# Autodesk Inventor assembly: Shoulder_Pitch_Assembly
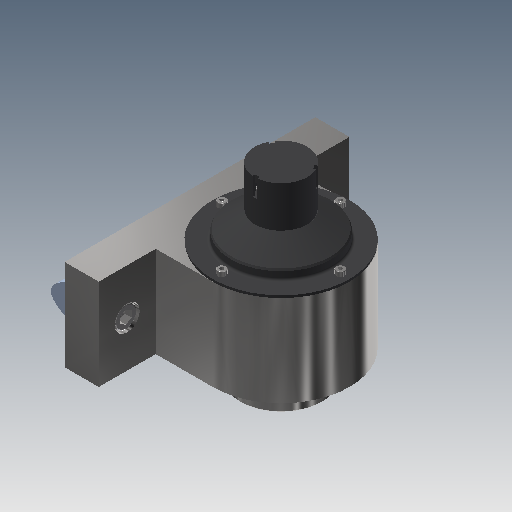
[picture p0: Inventor's stored thumbnail of the model, 512x512]
Saved by Autodesk Inventor 2021.4 (Build 254397000, 397)
## iProperties
Created: 2022-08-02
Part Number: Shoulder_Pitch_Assembly
Material: Generisch
Document SubType Name: Assembly
Designer: alexw
Mass: 1417.09 g
Surface Area: 710.967 cm^2
Volume: 192.324 cm^3
Density: 7.36827 g/cm^3
Author: alexw
## Documents named in this file (13)
- C:\Users\alexw\Documents\Inventor\Projects\03_CurrentProjects\MasterThesis\TrainingConsol_220422\Workgroups\Workgroup\Shoulder_Pitch_Assembly.iam
- C:\Users\alexw\Documents\Inventor\Projects\03_CurrentProjects\MasterThesis\TrainingConsol_220422\Workgroups\Workgroup\shoulder_joint_fit_v2.ipt
- C:\Users\alexw\Documents\Inventor\Projects\03_CurrentProjects\MasterThesis\TrainingConsol_220422\Workgroups\Workgroup\DIN 720 SKF - SKF 32005 X_Q.ipt
- C:\Users\alexw\Documents\Inventor\Projects\03_CurrentProjects\MasterThesis\TrainingConsol_220422\Workgroups\Workgroup\DIN 720 SKF - SKF 32004 X_Q.ipt
- C:\Users\alexw\Documents\Inventor\Projects\03_CurrentProjects\MasterThesis\TrainingConsol_220422\Workgroups\Workgroup\DIN EN ISO 7090 -  18.ipt
- C:\Users\alexw\Documents\Inventor\Projects\03_CurrentProjects\MasterThesis\TrainingConsol_220422\Workgroups\Workgroup\DIN 981 - KM 3.ipt
- C:\Users\alexw\Documents\Inventor\Projects\03_CurrentProjects\MasterThesis\TrainingConsol_220422\Workgroups\Workgroup\Shoulder_Shaft_Pitch.ipt
- C:\Users\alexw\Documents\Inventor\Projects\03_CurrentProjects\MasterThesis\TrainingConsol_220422\Workgroups\Workgroup\DIN EN ISO 4762 - M6 x 16.ipt
- C:\Users\alexw\Documents\Inventor\Projects\03_CurrentProjects\MasterThesis\TrainingConsol_220422\Workgroups\Workgroup\item_0038851_T-Slot_Nut_8_St_M6.ipt
- C:\Users\alexw\Documents\Inventor\Projects\03_CurrentProjects\MasterThesis\TrainingConsol_220422\Workgroups\Workgroup\Shoulder_Pitch_Sensor_Connector.ipt
- C:\Users\alexw\Documents\Inventor\Projects\03_CurrentProjects\MasterThesis\TrainingConsol_220422\Workgroups\Workgroup\Magnetic Encoder.ipt
- C:\Users\alexw\Documents\Inventor\Projects\03_CurrentProjects\MasterThesis\TrainingConsol_220422\Workgroups\Workgroup\DIN EN ISO 4762 - M2 x 8.ipt
- C:\Users\alexw\Documents\Inventor\Projects\03_CurrentProjects\MasterThesis\TrainingConsol_220422\Workgroups\Workgroup\DIN EN ISO 4762 - M2 x 6.ipt
## Components (18 placed, 12 different names)
1. shoulder_joint_fit_v2:1 — Mate:33, Flush:1, Mate:34, Mate:35, Angle:1, Angle:2
2. DIN 720 SKF- Präzision SKF 32005 X/Q:1
3. DIN 720 SKF- Präzision SKF 32004 X/Q:1
4. DIN EN ISO 7090 18:1
5. DIN 981 KM 3:1
6. Shoulder_Shaft_Pitch:1
7. DIN EN ISO 4762 M6 x 16:1 — Mate:37
8. DIN EN ISO 4762 M6 x 16:2 — Mate:36
9. Shoulder_Pitch_Sensor_Connector:1
10. Magnetic Encoder:1
11. DIN EN ISO 4762 M2 x 8:1
12. DIN EN ISO 4762 M2 x 8:2 — Mate:35
13. DIN EN ISO 4762 M2 x 8:3
14. DIN EN ISO 4762 M2 x 8:4
15. DIN EN ISO 4762 M2 x 6:1
16. DIN EN ISO 4762 M2 x 6:2
17. item_0038851_T-Slot_Nut_8_St_M6:1 — Mate:36, Angle:1, Flush:2
18. item_0038851_T-Slot_Nut_8_St_M6:2 — Mate:37, Angle:2, Flush:2
## Relationships (40: Mate 36, Flush 2, Angle 2)
- [Mate]: DIN 720 SKF- Präzision SKF 32004 X/Q:1 ↔ DIN EN ISO 7090 18:1
- [Mate]: DIN 720 SKF- Präzision SKF 32005 X/Q:1 ↔ Shoulder_Shaft_Pitch:1
- [Mate]: DIN EN ISO 7090 18:1 ↔ Shoulder_Shaft_Pitch:1
- [Mate]: DIN 981 KM 3:1 ↔ Shoulder_Shaft_Pitch:1
- [Mate]: DIN EN ISO 7090 18:1 ↔ DIN 981 KM 3:1
- [Mate]: shoulder_joint_fit_v2:1 ↔ Shoulder_Pitch_Sensor_Connector:1
- [Mate]: Shoulder_Pitch_Sensor_Connector:1 ↔ Magnetic Encoder:1
- [Mate]: Shoulder_Pitch_Sensor_Connector:1 ↔ DIN EN ISO 4762 M2 x 8:1
- [Mate]: Shoulder_Pitch_Sensor_Connector:1 ↔ DIN EN ISO 4762 M2 x 8:2
- [Mate]: Shoulder_Pitch_Sensor_Connector:1 ↔ DIN EN ISO 4762 M2 x 8:3
- [Mate]: Shoulder_Pitch_Sensor_Connector:1 ↔ DIN EN ISO 4762 M2 x 8:4
- [Mate]: Magnetic Encoder:1 ↔ DIN EN ISO 4762 M2 x 6:1
- [Mate]: Magnetic Encoder:1 ↔ DIN EN ISO 4762 M2 x 6:2
- [Mate]: DIN 720 SKF- Präzision SKF 32005 X/Q:1 ↔ Shoulder_Shaft_Pitch:1
- [Mate]: shoulder_joint_fit_v2:1 ↔ DIN EN ISO 4762 M6 x 16:2
- [Mate]: shoulder_joint_fit_v2:1 ↔ DIN EN ISO 4762 M6 x 16:2
- [Mate]: shoulder_joint_fit_v2:1 ↔ DIN EN ISO 4762 M6 x 16:1
- [Mate]: shoulder_joint_fit_v2:1 ↔ DIN EN ISO 4762 M6 x 16:1
- [Mate]: shoulder_joint_fit_v2:1 ↔ DIN 720 SKF- Präzision SKF 32005 X/Q:1
- [Mate]: DIN 720 SKF- Präzision SKF 32004 X/Q:1 ↔ Shoulder_Shaft_Pitch:1
- [Mate]: shoulder_joint_fit_v2:1 ↔ DIN 720 SKF- Präzision SKF 32004 X/Q:1
- [Mate]: shoulder_joint_fit_v2:1 ↔ Shoulder_Pitch_Sensor_Connector:1
- [Mate]: Shoulder_Pitch_Sensor_Connector:1 ↔ Magnetic Encoder:1
- [Mate]: shoulder_joint_fit_v2:1 ↔ Shoulder_Pitch_Sensor_Connector:1
- [Mate]: shoulder_joint_fit_v2:1 ↔ DIN EN ISO 4762 M2 x 8:1
- [Mate]: Shoulder_Pitch_Sensor_Connector:1 ↔ DIN EN ISO 4762 M2 x 8:4
- [Mate]: Shoulder_Pitch_Sensor_Connector:1 ↔ DIN EN ISO 4762 M2 x 8:3
- [Mate]: Shoulder_Pitch_Sensor_Connector:1 ↔ Magnetic Encoder:1
- [Mate]: Shoulder_Pitch_Sensor_Connector:1 ↔ DIN EN ISO 4762 M2 x 6:1
- [Mate]: Shoulder_Pitch_Sensor_Connector:1 ↔ DIN EN ISO 4762 M2 x 6:2
- [Mate]: shoulder_joint_fit_v2:1 ↔ Shoulder_Shaft_Pitch:1
- Mate:33: shoulder_joint_fit_v2:1
- Flush:1: shoulder_joint_fit_v2:1
- Mate:34: shoulder_joint_fit_v2:1
- Mate:35: shoulder_joint_fit_v2:1 ↔ DIN EN ISO 4762 M2 x 8:2
- Mate:36: DIN EN ISO 4762 M6 x 16:2 ↔ item_0038851_T-Slot_Nut_8_St_M6:1
- Angle:1 (0 deg): shoulder_joint_fit_v2:1 ↔ item_0038851_T-Slot_Nut_8_St_M6:1
- Mate:37: DIN EN ISO 4762 M6 x 16:1 ↔ item_0038851_T-Slot_Nut_8_St_M6:2
- Angle:2 (0 deg): shoulder_joint_fit_v2:1 ↔ item_0038851_T-Slot_Nut_8_St_M6:2
- Flush:2: item_0038851_T-Slot_Nut_8_St_M6:1 ↔ item_0038851_T-Slot_Nut_8_St_M6:2
## Named parameters: d326_d148 = 0 mm
